# Autodesk Inventor assembly: ASY DS-B beam 4
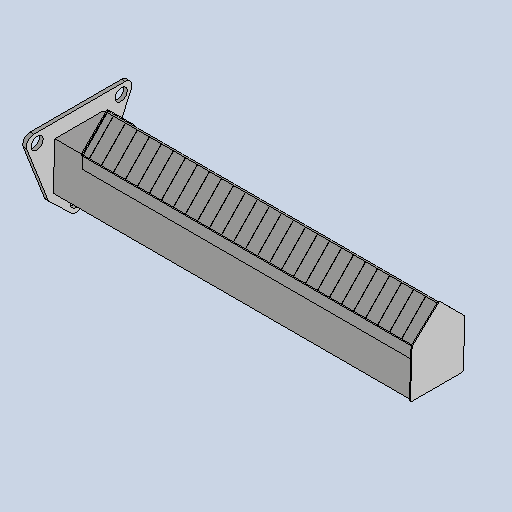
[picture p0: Inventor's stored thumbnail of the model, 512x512]
Saved by Autodesk Inventor 2025 (Build 290162010, 162A)
## iProperties
Created: 2025-02-18
Part Number: ASY DS-B beam 4
Document SubType Name: Assembly
Designer: admin
Author: admin
## Documents named in this file (6)
- C:\Users\admin\YandexDisk-badmisterfox\home pc\Inventor\filter-distribution-system\ASY DS-B beam 4.iam
- C:\Users\admin\YandexDisk-badmisterfox\home pc\Inventor\filter-distribution-system\DS-B-1101 beam 24.ipt
- C:\Users\admin\YandexDisk-badmisterfox\home pc\Inventor\filter-distribution-system\DS-B-1102 roof 24.ipt
- C:\Users\admin\YandexDisk-badmisterfox\home pc\Inventor\filter-distribution-system\DS-B-501 beam flange.ipt
- C:\Users\admin\YandexDisk-badmisterfox\home pc\Inventor\filter-distribution-system\DS-B-502 CAPhouse.ipt
- C:\Users\admin\YandexDisk-badmisterfox\home pc\Inventor\filter-distribution-system\DS-B-503 CAP.ipt
## Components (5 placed, 5 different names)
1. CDF-1101 beam 24:1 — Mate:2, Flush:3, Flush:4, Flush:1, Mate:1, Flush:6, Mate:6, Rigid:1, Rigid:2
2. CDF-1102 roof 24:1 — Flush:1, Mate:1, Flush:6, Mate:7
3. Part1:1 — Rigid:1
4. MNT-CDF-604 CAP:1 — Mate:3, Rigid:2
5. MNT-CDF-605 CAP:1 — Mate:5, Mate:6, Mate:7
## Relationships (12: Mate 6, Flush 4, WeldJoint 2)
- Mate:2: CDF-1101 beam 24:1
- Flush:3: CDF-1101 beam 24:1
- Flush:4: CDF-1101 beam 24:1
- Flush:1: CDF-1101 beam 24:1 ↔ CDF-1102 roof 24:1
- Mate:1: CDF-1101 beam 24:1 ↔ CDF-1102 roof 24:1
- Flush:6: CDF-1101 beam 24:1 ↔ CDF-1102 roof 24:1
- Mate:3: MNT-CDF-604 CAP:1
- Mate:5: MNT-CDF-605 CAP:1
- Mate:6: CDF-1101 beam 24:1 ↔ MNT-CDF-605 CAP:1
- Mate:7: CDF-1102 roof 24:1 ↔ MNT-CDF-605 CAP:1
- Rigid:1 [WeldJoint]: CDF-1101 beam 24:1 ↔ Part1:1
- Rigid:2 [WeldJoint]: CDF-1101 beam 24:1 ↔ MNT-CDF-604 CAP:1
